# Autodesk Inventor assembly: Chair
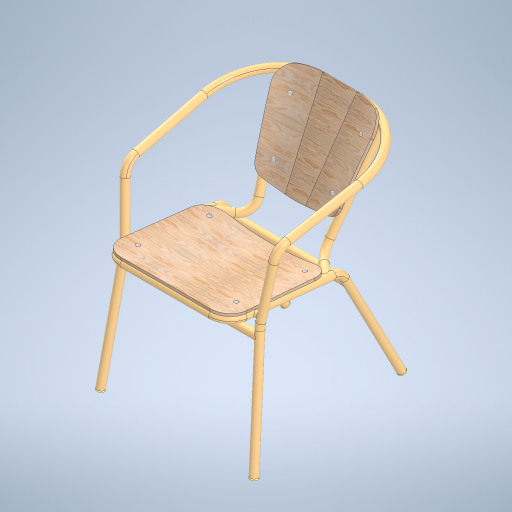
[picture p0: Inventor's stored thumbnail of the model, 512x512]
Saved by Autodesk Inventor 2024 (Build 280153000, 153)
## iProperties
Created: 2021-04-21
Part Number: Chair
Document SubType Name: Assembly
Designer: SauliusD
Author: SauliusD
## Documents named in this file (14)
- C:\W4INV 2024 Design\PROJECTS\Samples\Chair\Chair.iam
- C:\W4INV 2024 Design\PROJECTS\Samples\Chair\Parts\Front Leg.ipt
- C:\W4INV 2024 Design\PROJECTS\Samples\Chair\Parts\Seat Support and Back Leg.ipt
- C:\W4INV 2024 Design\PROJECTS\Samples\Chair\Parts\Back Rest support.ipt
- C:\W4INV 2024 Design\PROJECTS\Samples\Chair\Parts\Seat.ipt
- C:\W4INV 2024 Design\PROJECTS\Samples\Chair\Parts\Seat Back.ipt
- C:\W4INV 2024 Design\PROJECTS\Samples\Chair\Parts\Front support.ipt
- C:\W4INV 2024 Design\PROJECTS\Samples\Chair\Parts\Back support.ipt
- C:\W4INV 2024 Design\PROJECTS\Samples\Chair\Parts\Joint.ipt
- C:\W4INV 2024 Design\PROJECTS\Samples\Chair\Parts\Back Rest support_MIR.ipt
- C:\W4INV 2024 Design\PROJECTS\Samples\Chair\Parts\Joint_MIR.ipt
- C:\W4INV 2024 Design\PROJECTS\Samples\Chair\Parts\Front Seat fixture.ipt
- C:\W4INV 2024 Design\PROJECTS\Samples\Chair\Parts\Filler Cap.ipt
- C:\W4INV 2024 Design\PROJECTS\Samples\Chair\Parts\Rivet.ipt
## Components (30 placed, 13 different names)
1. Front Leg:1 — Flush:1, Flush:2, Flush:3, Insert:1, Insert:4, Flush:17, Flush:18, Flush:19, Mate:10, Flush:20, Flush:21
2. Seat Support and Back Leg:1 — Flush:4, Flush:5, Flush:6, Mate:3, Mate:4, Mate:5, Insert:2, Insert:3
3. Back Rest support:1 — Flush:7, Flush:8, Flush:9, Mate:7, Mate:8
4. Seat:1 — Flush:10, Flush:11, Flush:12
5. Seat Back:1 — Flush:13, Flush:14, Flush:15
6. Front support:1
7. Back support:1
8. Joint:1
9. Back Rest support_MIR:1 — Mate:1, Flush:16, Mate:2, Mate:6, Mate:9
10. Joint_MIR:1
11. Front Seat fixture:1 — Insert:7, Symmetry:3
12. Front Seat fixture:2 — Mate:3, Insert:5, Flush:20, Symmetry:4
13. Front Seat fixture:3 — Mate:4, Insert:8, Mate:10, Symmetry:3
14. Front Seat fixture:4 — Mate:5, Insert:6, Flush:21, Symmetry:4
15. Front Seat fixture:5 — Mate:6, Insert:10, Symmetry:1
16. Front Seat fixture:6 — Mate:7, Insert:9, Flush:17, Symmetry:1
17. Filler Cap:2 — Insert:2
18. Filler Cap:3 — Insert:1
19. Filler Cap:4 — Insert:4
20. Filler Cap:5 — Insert:3
21. Rivet:2 — Insert:6
22. Rivet:3 — Insert:5
23. Rivet:4 — Insert:8
24. Rivet:5 — Insert:7
25. Rivet:6 — Insert:10
26. Rivet:7 — Insert:9
27. Front Seat fixture:7 — Mate:8, Flush:18, Symmetry:2, Insert:12
28. Front Seat fixture:8 — Mate:9, Flush:19, Symmetry:2, Insert:11
29. Rivet:8 — Insert:12
30. Rivet:9 — Insert:11
## Relationships (47: Flush 21, Insert 12, Mate 10, Symmetry 4)
- Flush:1: Front Leg:1
- Flush:2: Front Leg:1
- Flush:3: Front Leg:1
- Flush:4: Seat Support and Back Leg:1
- Flush:5: Seat Support and Back Leg:1
- Flush:6: Seat Support and Back Leg:1
- Flush:7: Back Rest support:1
- Flush:8: Back Rest support:1
- Flush:9: Back Rest support:1
- Flush:10: Seat:1
- Flush:11: Seat:1
- Flush:12: Seat:1
- Flush:13: Seat Back:1
- Flush:14: Seat Back:1
- Flush:15: Seat Back:1
- Mate:1: Back Rest support_MIR:1
- Flush:16: Back Rest support_MIR:1
- Mate:2: Back Rest support_MIR:1
- Mate:3: Seat Support and Back Leg:1 ↔ Front Seat fixture:2
- Mate:4: Seat Support and Back Leg:1 ↔ Front Seat fixture:3
- Mate:5: Seat Support and Back Leg:1 ↔ Front Seat fixture:4
- Mate:6: Back Rest support_MIR:1 ↔ Front Seat fixture:5
- Mate:7: Back Rest support:1 ↔ Front Seat fixture:6
- Insert:2: Seat Support and Back Leg:1 ↔ Filler Cap:2
- Insert:1: Front Leg:1 ↔ Filler Cap:3
- Insert:4: Front Leg:1 ↔ Filler Cap:4
- Insert:3: Seat Support and Back Leg:1 ↔ Filler Cap:5
- Insert:6: Front Seat fixture:4 ↔ Rivet:2
- Insert:5: Front Seat fixture:2 ↔ Rivet:3
- Insert:8: Front Seat fixture:3 ↔ Rivet:4
- Insert:7: Front Seat fixture:1 ↔ Rivet:5
- Insert:10: Front Seat fixture:5 ↔ Rivet:6
- Insert:9: Front Seat fixture:6 ↔ Rivet:7
- Flush:17: Front Leg:1 ↔ Front Seat fixture:6
- Symmetry:1: Front Seat fixture:5 ↔ Front Seat fixture:6
- Mate:8: Back Rest support:1 ↔ Front Seat fixture:7
- Mate:9: Back Rest support_MIR:1 ↔ Front Seat fixture:8
- Flush:18: Front Leg:1 ↔ Front Seat fixture:7
- Flush:19: Front Leg:1 ↔ Front Seat fixture:8
- Symmetry:2: Front Seat fixture:7 ↔ Front Seat fixture:8
- Insert:12: Front Seat fixture:7 ↔ Rivet:8
- Insert:11: Front Seat fixture:8 ↔ Rivet:9
- Mate:10: Front Leg:1 ↔ Front Seat fixture:3
- Symmetry:3: Front Seat fixture:1 ↔ Front Seat fixture:3
- Flush:20: Front Leg:1 ↔ Front Seat fixture:2
- Flush:21: Front Leg:1 ↔ Front Seat fixture:4
- Symmetry:4: Front Seat fixture:2 ↔ Front Seat fixture:4
